# Autodesk Inventor assembly: leg_Left_femur_ass
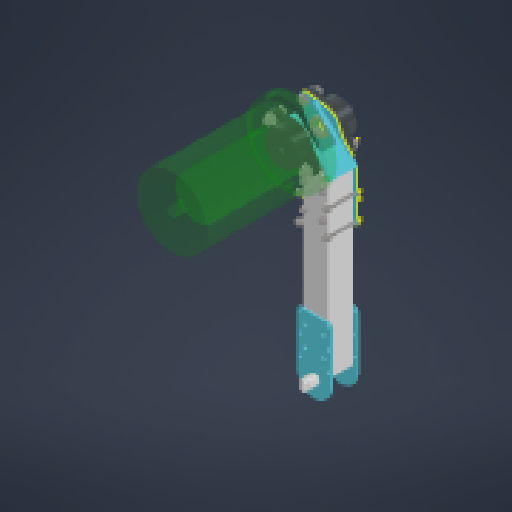
[picture p0: Inventor's stored thumbnail of the model, 512x512]
Saved by Autodesk Inventor 2026 (Build 300175000, 175)
## iProperties
Created: 2026-04-24
Part Number: leg_Left_femur_ass
Document SubType Name: Assembly
Designer: user
Mass: 1158.5 g
Surface Area: 2231.02 cm^2
Volume: 319.422 cm^3
Author: user
## Documents named in this file (14)
- C:\Users\user\vs_code_projects\ogonek-spider\physical-structure\cad\leg_femur\leg_Right_femur_ass.iam
- C:\Users\user\vs_code_projects\ogonek-spider\physical-structure\cad\leg_femur\femur_profile.ipt
- C:\Users\user\vs_code_projects\ogonek-spider\physical-structure\cad\leg_femur\femur_support_steel.ipt
- C:\Users\user\vs_code_projects\ogonek-spider\physical-structure\cad\leg_femur\femur_motor_steel.ipt
- C:\Users\user\vs_code_projects\ogonek-spider\physical-structure\cad\leg_femur\femur_outside_steel.ipt
- C:\Users\user\vs_code_projects\ogonek-spider\physical-structure\cad\leg_femur\shaft_femur.ipt
- C:\Users\user\vs_code_projects\ogonek-spider\physical-structure\cad\body_parts\motor_mass.ipt
- C:\Users\user\vs_code_projects\ogonek-spider\physical-structure\cad\leg_femur\femur_reinforcement_tibea_steel.ipt
- C:\Users\user\Documents\Inventor\Content Center Files\R2026\ru-RU\GOST 10338-80\Винт M10-6gx32 ГОСТ 10338-80.ipt
- C:\Users\user\Documents\Inventor\Content Center Files\R2026\ru-RU\Nut GOST R ISO 4161-2013\ГайкаM10-6H ГОСТ Р ISO 4161-2013.ipt
- C:\Users\user\Documents\Inventor\Content Center Files\R2026\ru-RU\Bolt 2 GOST 15591-70\Болт 2 M6×65 ГОСТ 15591-70.ipt
- C:\Users\user\Documents\Inventor\Content Center Files\R2026\ru-RU\Nut GOST R ISO 4161-2013\ГайкаM6-6H ГОСТ Р ISO 4161-2013.ipt
- C:\Users\user\Documents\Inventor\Content Center Files\R2026\ru-RU\GOST 7872-89 (8000H)\Подшипник 8104H ГОСТ 7872-89.ipt
- C:\Users\user\vs_code_projects\ogonek-spider\physical-structure\cad\screw\bearing_unit_20mm.ipt
## Components (44 placed, 13 different names)
1. femur_profile:1 — Жесткий:2, Жесткий:3, С поворотом:1, С поворотом:2, С поворотом:3, С поворотом:4
2. femur_support_steel:1 — С поворотом:1, С поворотом:2, Жесткий:6, Совмещение:17, Совмещение:18, Совмещение:19, Совмещение:20, Совмещение:21, Совмещение:22, Совмещение:23, Совмещение:24, Совмещение:25, Совмещение:26, Совмещение:27, Совмещение:28, Совмещение:29, Совмещение:30, Совмещение:31, Совмещение:32, Совмещение:33, Совмещение:35, Совмещение:37, Совмещение:39, Совмещение:41, Совмещение:43, Совмещение:45, Совмещение:47, Вставка:2, С поворотом:17, С поворотом:18, Совмещение:65, Совмещение:66, Совмещение:67, Совмещение:68, Совмещение:69, Совмещение:70, Совмещение:71, Совмещение:72, Совмещение:73, Совмещение:75, Совмещение:77, Совмещение:79
3. femur_motor_steel:1 — С поворотом:3, С поворотом:4, С поворотом:15, С поворотом:16, Совмещение:34, Совмещение:36, Совмещение:38, Совмещение:40, Совмещение:42, Совмещение:44, Совмещение:46, Совмещение:48, Вставка:1, С поворотом:19, С поворотом:20, Совмещение:49, Совмещение:50, Совмещение:51, Совмещение:52, Совмещение:54, Совмещение:55, Совмещение:56, Совмещение:57, Совмещение:59, Совмещение:63
4. femur_outside_steel:1 — Жесткий:2
5. femur_outside_steel:2 — Жесткий:3, Жесткий:5
6. shaft_femur:1 — Жесткий:5
7. motor_mass:1 — С поворотом:15, С поворотом:16
8. femur_reinforcement_tibea_steel:1 — Жесткий:6
9. Подшипник 8000H ГОСТ 7872-89 8104H:1 — Вставка:1
10. Подшипник 8000H ГОСТ 7872-89 8104H:2 — Вставка:2
11. bearing_unit_20mm:1 — С поворотом:17, С поворотом:18, Совмещение:74, Совмещение:76, Совмещение:78, Совмещение:80
12. bearing_unit_20mm:2 — С поворотом:19, С поворотом:20, Совмещение:53, Совмещение:58, Совмещение:60, Совмещение:61, Совмещение:62, Совмещение:64
13. Винт ГОСТ 10338-80 M 10 x 32:1 — Совмещение:49, Совмещение:50
14. Гайка ГОСТ Р ISO 4161-2013 M10:1 — Совмещение:57, Совмещение:58
15. Винт ГОСТ 10338-80 M 10 x 32:2 — Совмещение:51, Совмещение:52
16. Винт ГОСТ 10338-80 M 10 x 32:3 — Совмещение:53, Совмещение:54
17. Винт ГОСТ 10338-80 M 10 x 32:4 — Совмещение:55, Совмещение:56
18. Гайка ГОСТ Р ISO 4161-2013 M10:2 — Совмещение:59, Совмещение:60
19. Гайка ГОСТ Р ISO 4161-2013 M10:3 — Совмещение:61, Совмещение:62
20. Гайка ГОСТ Р ISO 4161-2013 M10:4 — Совмещение:63, Совмещение:64
21. Винт ГОСТ 10338-80 M 10 x 32:5 — Совмещение:65, Совмещение:66
22. Гайка ГОСТ Р ISO 4161-2013 M10:5 — Совмещение:73, Совмещение:74
23. Винт ГОСТ 10338-80 M 10 x 32:6 — Совмещение:67, Совмещение:68
24. Винт ГОСТ 10338-80 M 10 x 32:7 — Совмещение:69, Совмещение:70
25. Винт ГОСТ 10338-80 M 10 x 32:8 — Совмещение:71, Совмещение:72
26. Гайка ГОСТ Р ISO 4161-2013 M10:6 — Совмещение:75, Совмещение:76
27. Гайка ГОСТ Р ISO 4161-2013 M10:7 — Совмещение:77, Совмещение:78
28. Гайка ГОСТ Р ISO 4161-2013 M10:8 — Совмещение:79, Совмещение:80
29. Болт 2 ГОСТ 15591-70 M6×65:1 — Совмещение:17, Совмещение:18
30. Гайка ГОСТ Р ISO 4161-2013 M6:1 — Совмещение:33, Совмещение:34
31. Болт 2 ГОСТ 15591-70 M6×65:2 — Совмещение:19, Совмещение:20
32. Болт 2 ГОСТ 15591-70 M6×65:3 — Совмещение:21, Совмещение:22
33. Болт 2 ГОСТ 15591-70 M6×65:4 — Совмещение:23, Совмещение:24
34. Болт 2 ГОСТ 15591-70 M6×65:5 — Совмещение:25, Совмещение:26
35. Болт 2 ГОСТ 15591-70 M6×65:6 — Совмещение:27, Совмещение:28
36. Болт 2 ГОСТ 15591-70 M6×65:7 — Совмещение:29, Совмещение:30
37. Болт 2 ГОСТ 15591-70 M6×65:8 — Совмещение:31, Совмещение:32
38. Гайка ГОСТ Р ISO 4161-2013 M6:2 — Совмещение:35, Совмещение:36
39. Гайка ГОСТ Р ISO 4161-2013 M6:3 — Совмещение:37, Совмещение:38
40. Гайка ГОСТ Р ISO 4161-2013 M6:4 — Совмещение:39, Совмещение:40
41. Гайка ГОСТ Р ISO 4161-2013 M6:5 — Совмещение:41, Совмещение:42
42. Гайка ГОСТ Р ISO 4161-2013 M6:6 — Совмещение:43, Совмещение:44
43. Гайка ГОСТ Р ISO 4161-2013 M6:7 — Совмещение:45, Совмещение:46
44. Гайка ГОСТ Р ISO 4161-2013 M6:8 — Совмещение:47, Совмещение:48
## Relationships (80: Mate 64, RevoluteJoint 10, WeldJoint 4, Insert 2)
- Жесткий:2 [WeldJoint]: femur_profile:1 ↔ femur_outside_steel:1
- Жесткий:3 [WeldJoint]: femur_profile:1 ↔ femur_outside_steel:2
- Жесткий:5 [WeldJoint] (20 mm): femur_outside_steel:2 ↔ shaft_femur:1
- С поворотом:1 [RevoluteJoint]: femur_profile:1 ↔ femur_support_steel:1
- С поворотом:2 [RevoluteJoint]: femur_profile:1 ↔ femur_support_steel:1
- С поворотом:3 [RevoluteJoint]: femur_profile:1 ↔ femur_motor_steel:1
- С поворотом:4 [RevoluteJoint]: femur_profile:1 ↔ femur_motor_steel:1
- С поворотом:15 [RevoluteJoint]: femur_motor_steel:1 ↔ motor_mass:1
- С поворотом:16 [RevoluteJoint]: femur_motor_steel:1 ↔ motor_mass:1
- Жесткий:6 [WeldJoint]: femur_support_steel:1 ↔ femur_reinforcement_tibea_steel:1
- Совмещение:17 [Mate]: femur_support_steel:1 ↔ Болт 2 ГОСТ 15591-70 M6×65:1
- Совмещение:18 [Mate]: femur_support_steel:1 ↔ Болт 2 ГОСТ 15591-70 M6×65:1
- Совмещение:19 [Mate]: femur_support_steel:1 ↔ Болт 2 ГОСТ 15591-70 M6×65:2
- Совмещение:20 [Mate]: femur_support_steel:1 ↔ Болт 2 ГОСТ 15591-70 M6×65:2
- Совмещение:21 [Mate]: femur_support_steel:1 ↔ Болт 2 ГОСТ 15591-70 M6×65:3
- Совмещение:22 [Mate]: femur_support_steel:1 ↔ Болт 2 ГОСТ 15591-70 M6×65:3
- Совмещение:23 [Mate]: femur_support_steel:1 ↔ Болт 2 ГОСТ 15591-70 M6×65:4
- Совмещение:24 [Mate]: femur_support_steel:1 ↔ Болт 2 ГОСТ 15591-70 M6×65:4
- Совмещение:25 [Mate]: femur_support_steel:1 ↔ Болт 2 ГОСТ 15591-70 M6×65:5
- Совмещение:26 [Mate]: femur_support_steel:1 ↔ Болт 2 ГОСТ 15591-70 M6×65:5
- Совмещение:27 [Mate]: femur_support_steel:1 ↔ Болт 2 ГОСТ 15591-70 M6×65:6
- Совмещение:28 [Mate]: femur_support_steel:1 ↔ Болт 2 ГОСТ 15591-70 M6×65:6
- Совмещение:29 [Mate]: femur_support_steel:1 ↔ Болт 2 ГОСТ 15591-70 M6×65:7
- Совмещение:30 [Mate]: femur_support_steel:1 ↔ Болт 2 ГОСТ 15591-70 M6×65:7
- Совмещение:31 [Mate]: femur_support_steel:1 ↔ Болт 2 ГОСТ 15591-70 M6×65:8
- Совмещение:32 [Mate]: femur_support_steel:1 ↔ Болт 2 ГОСТ 15591-70 M6×65:8
- Совмещение:33 [Mate]: femur_support_steel:1 ↔ Гайка ГОСТ Р ISO 4161-2013 M6:1
- Совмещение:34 [Mate]: femur_motor_steel:1 ↔ Гайка ГОСТ Р ISO 4161-2013 M6:1
- Совмещение:35 [Mate]: femur_support_steel:1 ↔ Гайка ГОСТ Р ISO 4161-2013 M6:2
- Совмещение:36 [Mate]: femur_motor_steel:1 ↔ Гайка ГОСТ Р ISO 4161-2013 M6:2
- Совмещение:37 [Mate]: femur_support_steel:1 ↔ Гайка ГОСТ Р ISO 4161-2013 M6:3
- Совмещение:38 [Mate]: femur_motor_steel:1 ↔ Гайка ГОСТ Р ISO 4161-2013 M6:3
- Совмещение:39 [Mate]: femur_support_steel:1 ↔ Гайка ГОСТ Р ISO 4161-2013 M6:4
- Совмещение:40 [Mate]: femur_motor_steel:1 ↔ Гайка ГОСТ Р ISO 4161-2013 M6:4
- Совмещение:41 [Mate]: femur_support_steel:1 ↔ Гайка ГОСТ Р ISO 4161-2013 M6:5
- Совмещение:42 [Mate]: femur_motor_steel:1 ↔ Гайка ГОСТ Р ISO 4161-2013 M6:5
- Совмещение:43 [Mate]: femur_support_steel:1 ↔ Гайка ГОСТ Р ISO 4161-2013 M6:6
- Совмещение:44 [Mate]: femur_motor_steel:1 ↔ Гайка ГОСТ Р ISO 4161-2013 M6:6
- Совмещение:45 [Mate]: femur_support_steel:1 ↔ Гайка ГОСТ Р ISO 4161-2013 M6:7
- Совмещение:46 [Mate]: femur_motor_steel:1 ↔ Гайка ГОСТ Р ISO 4161-2013 M6:7
- Совмещение:47 [Mate]: femur_support_steel:1 ↔ Гайка ГОСТ Р ISO 4161-2013 M6:8
- Совмещение:48 [Mate]: femur_motor_steel:1 ↔ Гайка ГОСТ Р ISO 4161-2013 M6:8
- Вставка:1 [Insert]: femur_motor_steel:1 ↔ Подшипник 8000H ГОСТ 7872-89 8104H:1
- Вставка:2 [Insert]: femur_support_steel:1 ↔ Подшипник 8000H ГОСТ 7872-89 8104H:2
- С поворотом:17 [RevoluteJoint]: femur_support_steel:1 ↔ bearing_unit_20mm:1
- С поворотом:18 [RevoluteJoint]: femur_support_steel:1 ↔ bearing_unit_20mm:1
- С поворотом:19 [RevoluteJoint]: femur_motor_steel:1 ↔ bearing_unit_20mm:2
- С поворотом:20 [RevoluteJoint]: femur_motor_steel:1 ↔ bearing_unit_20mm:2
- Совмещение:49 [Mate]: femur_motor_steel:1 ↔ Винт ГОСТ 10338-80 M 10 x 32:1
- Совмещение:50 [Mate]: femur_motor_steel:1 ↔ Винт ГОСТ 10338-80 M 10 x 32:1
- Совмещение:51 [Mate]: femur_motor_steel:1 ↔ Винт ГОСТ 10338-80 M 10 x 32:2
- Совмещение:52 [Mate]: femur_motor_steel:1 ↔ Винт ГОСТ 10338-80 M 10 x 32:2
- Совмещение:53 [Mate]: bearing_unit_20mm:2 ↔ Винт ГОСТ 10338-80 M 10 x 32:3
- Совмещение:54 [Mate]: femur_motor_steel:1 ↔ Винт ГОСТ 10338-80 M 10 x 32:3
- Совмещение:55 [Mate]: femur_motor_steel:1 ↔ Винт ГОСТ 10338-80 M 10 x 32:4
- Совмещение:56 [Mate]: femur_motor_steel:1 ↔ Винт ГОСТ 10338-80 M 10 x 32:4
- Совмещение:57 [Mate]: femur_motor_steel:1 ↔ Гайка ГОСТ Р ISO 4161-2013 M10:1
- Совмещение:58 [Mate]: bearing_unit_20mm:2 ↔ Гайка ГОСТ Р ISO 4161-2013 M10:1
- Совмещение:59 [Mate]: femur_motor_steel:1 ↔ Гайка ГОСТ Р ISO 4161-2013 M10:2
- Совмещение:60 [Mate]: bearing_unit_20mm:2 ↔ Гайка ГОСТ Р ISO 4161-2013 M10:2
- Совмещение:61 [Mate]: bearing_unit_20mm:2 ↔ Гайка ГОСТ Р ISO 4161-2013 M10:3
- Совмещение:62 [Mate]: bearing_unit_20mm:2 ↔ Гайка ГОСТ Р ISO 4161-2013 M10:3
- Совмещение:63 [Mate]: femur_motor_steel:1 ↔ Гайка ГОСТ Р ISO 4161-2013 M10:4
- Совмещение:64 [Mate]: bearing_unit_20mm:2 ↔ Гайка ГОСТ Р ISO 4161-2013 M10:4
- Совмещение:65 [Mate]: femur_support_steel:1 ↔ Винт ГОСТ 10338-80 M 10 x 32:5
- Совмещение:66 [Mate]: femur_support_steel:1 ↔ Винт ГОСТ 10338-80 M 10 x 32:5
- Совмещение:67 [Mate]: femur_support_steel:1 ↔ Винт ГОСТ 10338-80 M 10 x 32:6
- Совмещение:68 [Mate]: femur_support_steel:1 ↔ Винт ГОСТ 10338-80 M 10 x 32:6
- Совмещение:69 [Mate]: femur_support_steel:1 ↔ Винт ГОСТ 10338-80 M 10 x 32:7
- Совмещение:70 [Mate]: femur_support_steel:1 ↔ Винт ГОСТ 10338-80 M 10 x 32:7
- Совмещение:71 [Mate]: femur_support_steel:1 ↔ Винт ГОСТ 10338-80 M 10 x 32:8
- Совмещение:72 [Mate]: femur_support_steel:1 ↔ Винт ГОСТ 10338-80 M 10 x 32:8
- Совмещение:73 [Mate]: femur_support_steel:1 ↔ Гайка ГОСТ Р ISO 4161-2013 M10:5
- Совмещение:74 [Mate]: bearing_unit_20mm:1 ↔ Гайка ГОСТ Р ISO 4161-2013 M10:5
- Совмещение:75 [Mate]: femur_support_steel:1 ↔ Гайка ГОСТ Р ISO 4161-2013 M10:6
- Совмещение:76 [Mate]: bearing_unit_20mm:1 ↔ Гайка ГОСТ Р ISO 4161-2013 M10:6
- Совмещение:77 [Mate]: femur_support_steel:1 ↔ Гайка ГОСТ Р ISO 4161-2013 M10:7
- Совмещение:78 [Mate]: bearing_unit_20mm:1 ↔ Гайка ГОСТ Р ISO 4161-2013 M10:7
- Совмещение:79 [Mate]: femur_support_steel:1 ↔ Гайка ГОСТ Р ISO 4161-2013 M10:8
- Совмещение:80 [Mate]: bearing_unit_20mm:1 ↔ Гайка ГОСТ Р ISO 4161-2013 M10:8
